# Autodesk Inventor assembly: 24563131
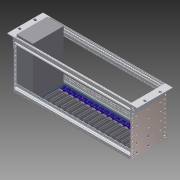
[picture p0: Inventor's stored thumbnail of the model, 180x180]
Saved by Autodesk Inventor 2015 (Build 190159000, 159)
## iProperties
Company: TraceParts S.A.
Created: 2014-08-14
Part Number: 24563131
Checked By: TraceParts S.A.
Catalog Web Link: www.traceparts.com
Document SubType Name: Assembly
Designer: TraceParts
Author: TraceParts
## Documents named in this file (29)
- C:\Users\smkilani\Documents\GitHub\G-2\LVBackplane\3D\24563131.iam
- C:\Users\smkilani\Downloads\24563131\24563131_26.ipt
- C:\Users\smkilani\Downloads\24563131\24563131_25.ipt
- C:\Users\smkilani\Downloads\24563131\24563131_24.ipt
- C:\Users\smkilani\Downloads\24563131\24563131_23.ipt
- C:\Users\smkilani\Downloads\24563131\24563131_22.ipt
- C:\Users\smkilani\Downloads\24563131\24563131_21.ipt
- C:\Users\smkilani\Downloads\24563131\24563131_20.ipt
- C:\Users\smkilani\Downloads\24563131\24563131_19.ipt
- C:\Users\smkilani\Downloads\24563131\24563131_18.ipt
- C:\Users\smkilani\Downloads\24563131\24563131_17.ipt
- C:\Users\smkilani\Downloads\24563131\24563131_16.ipt
- C:\Users\smkilani\Downloads\24563131\24563131_15.ipt
- C:\Users\smkilani\Downloads\24563131\24563131_14.ipt
- C:\Users\smkilani\Downloads\24563131\24563131_13.ipt
- C:\Users\smkilani\Downloads\24563131\24563131_12.ipt
- C:\Users\smkilani\Downloads\24563131\24563131_11.ipt
- C:\Users\smkilani\Downloads\24563131\24563131_10.ipt
- C:\Users\smkilani\Downloads\24563131\24563131_09.ipt
- C:\Users\smkilani\Downloads\24563131\24563131_08.ipt
- C:\Users\smkilani\Downloads\24563131\24563131_07.ipt
- C:\Users\smkilani\Downloads\24563131\24563131_06.ipt
- C:\Users\smkilani\Downloads\24563131\24563131_05.ipt
- C:\Users\smkilani\Downloads\24563131\24563131_04.ipt
- C:\Users\smkilani\Downloads\24563131\24563131_03.ipt
- C:\Users\smkilani\Downloads\24563131\24563131_02.ipt
- C:\Users\smkilani\Downloads\24563131\24563131_01.ipt
- C:\Users\smkilani\Documents\GitHub\G-2\LVBackplane\3D\PSU.ipt
- C:\Users\smkilani\Documents\GitHub\G-2\LVBackplane\3D\Imported Components\Backplane2\Backplane2.iam
## Components (28 placed, 28 different names)
1. 24563131_26:1
2. 24563131_25:1
3. 24563131_24:1
4. 24563131_23:1
5. 24563131_22:1
6. 24563131_21:1
7. 24563131_20:1
8. 24563131_19:1
9. 24563131_18:1
10. 24563131_17:1
11. 24563131_16:1
12. 24563131_15:1
13. 24563131_14:1 — Rigid:1
14. 24563131_13:1
15. 24563131_12:1 — Rotational:1
16. 24563131_11:1
17. 24563131_10:1
18. 24563131_09:1
19. 24563131_08:1
20. 24563131_07:1
21. 24563131_06:1
22. 24563131_05:1
23. 24563131_04:1
24. 24563131_03:1
25. 24563131_02:1
26. 24563131_01:1
27. PSU:1 — Rigid:1
28. Backplane2:1 [sub-assembly] — Rotational:1
## Relationships (2: WeldJoint 1, RevoluteJoint 1)
- Rigid:1 [WeldJoint]: 24563131_14:1 ↔ PSU:1
- Rotational:1 [RevoluteJoint] (1 mm): 24563131_12:1 ↔ Backplane2:1
